# Autodesk Inventor assembly: X-Gantry Joiner Right V3 Assembly
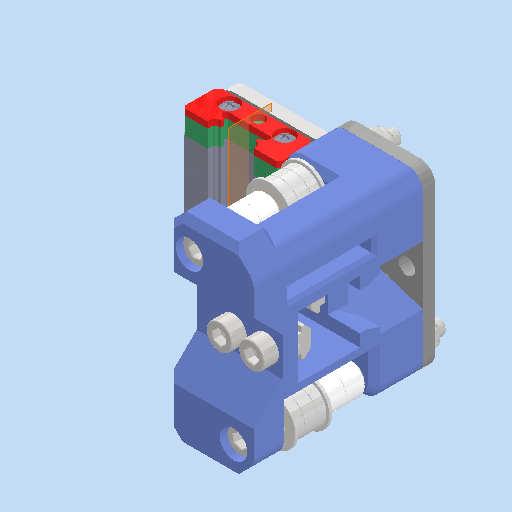
[picture p0: Inventor's stored thumbnail of the model, 512x512]
Saved by Autodesk Inventor 2023.2 (Build 272271000, 271)
## iProperties
Created: 2023-12-06
Part Number: X-Gantry Joiner Right V3 Assembly
Document SubType Name: Assembly
Designer: Nils Bade
Author: Nils Bade
## Documents named in this file (13)
- C:\Users\nilsb\Documents\Inventor\Projektarbeit-Bade\RatRig_Bade\X-Gantry Joiner Right V3 Assembly.iam
- C:\Users\nilsb\Documents\Inventor\Projektarbeit-Bade\RatRig_modified\xy Joiner Right for 4040 V2.ipt
- C:\Users\nilsb\Documents\Inventor\Projektarbeit-Bade\RatRig_modified\MGN15 Linear-Rail-Block.ipt
- C:\Users\nilsb\Documents\Inventor\Projektarbeit-Bade\Schrauben\Cap Head Screw M3x12 v2.ipt
- C:\Users\nilsb\Documents\Inventor\Projektarbeit-Bade\RatRig_Standards\T-Nut - Square type for 2020 - M5 v2.ipt
- C:\Users\nilsb\Documents\Inventor\Projektarbeit-Bade\Schrauben\Cap Head Screw M5x10 v2.ipt
- C:\Users\nilsb\Documents\Inventor\Projektarbeit-Bade\Schrauben\Cap Head Screw M5x60.ipt
- C:\Users\nilsb\Documents\Inventor\Projektarbeit-Bade\RatRig_Standards\Hex Locking Nut - M5 v2.ipt
- C:\Users\nilsb\Documents\Inventor\Projektarbeit-Bade\RatRig_Standards\Mini Precision Shim - 8x5x1mm v2.ipt
- C:\Users\nilsb\Documents\Inventor\Projektarbeit-Bade\RatRig_Standards\Ball Bearing - F695ZZ v1.ipt
- C:\Users\nilsb\Documents\Inventor\Projektarbeit-Bade\RatRig_Standards\Ball Bearing - 695ZZ v1.ipt
- C:\Users\nilsb\Documents\Inventor\Projektarbeit-Bade\RatRig_Standards\Aluminium Spacer - 6mm v2.ipt
- C:\Users\nilsb\Documents\Inventor\Projektarbeit-Bade\RatRig_modified\XY Joiner Plate for 4040 V1.ipt
## Components (33 placed, 12 different names)
1. xy Joiner Right for 4040 V2:1 — Passend:63, Passend:65, Passend:66, Passend:67, Passend:68, Passend:70, Passend:71, Passend:72, Passend:74, Passend:75, Passend:76, Passend:79, Passend:80, Passend:81, Passend:82
2. XY Joiner Plate for 4040 V1:2
3. MGN15 Linear-Rail-Block:1
4. Cap Head Screw M3x12 v2:1
5. Cap Head Screw M3x12 v2:2
6. Cap Head Screw M3x12 v2:3
7. Cap Head Screw M3x12 v2:4
8. T-Nut - Square type for 2020 - M5 v2:1 — Passend:73, Passend:74
9. T-Nut - Square type for 2020 - M5 v2:2 — Passend:78, Passend:80
10. T-Nut - Square type for 2020 - M5 v2:3 — Passend:77, Passend:79
11. Cap Head Screw M5x10 v2:1 — Passend:75, Passend:78, Passend:82
12. Cap Head Screw M5x10 v2:2 — Passend:76, Passend:77, Passend:81
13. Cap Head Screw M5x60:1 — Passend:63, Passend:66
14. Cap Head Screw M5x60:2 — Passend:67, Passend:70
15. Hex Locking Nut - M5 v2:1
16. Hex Locking Nut - M5 v2:2
17. Mini Precision Shim - 8x5x1mm v2:1
18. Mini Precision Shim - 8x5x1mm v2:2
19. Mini Precision Shim - 8x5x1mm v2:3 — Passend:68
20. Mini Precision Shim - 8x5x1mm v2:4
21. Mini Precision Shim - 8x5x1mm v2:5
22. Mini Precision Shim - 8x5x1mm v2:6 — Passend:65
23. Ball Bearing - F695ZZ v1:1
24. Ball Bearing - F695ZZ v1:2
25. Ball Bearing - F695ZZ v1:3
26. Ball Bearing - F695ZZ v1:4
27. Ball Bearing - 695ZZ v1:1
28. Ball Bearing - 695ZZ v1:2
29. Aluminium Spacer - 6mm v2:1
30. Aluminium Spacer - 6mm v2:2
31. Aluminium Spacer - 6mm v2:3
32. Aluminium Spacer - 6mm v2:4
33. Cap Head Screw M5x10 v2:3 — Passend:71, Passend:72, Passend:73
## Relationships (68: Mate 68)
- [Mate]: Cap Head Screw M5x60:1 ↔ Hex Locking Nut - M5 v2:1
- [Mate]: Cap Head Screw M5x60:2 ↔ Hex Locking Nut - M5 v2:2
- [Mate]: Cap Head Screw M5x60:2 ↔ Mini Precision Shim - 8x5x1mm v2:3
- [Mate]: Cap Head Screw M5x60:2 ↔ Ball Bearing - F695ZZ v1:4
- [Mate]: Mini Precision Shim - 8x5x1mm v2:3 ↔ Ball Bearing - F695ZZ v1:4
- [Mate]: Cap Head Screw M5x60:2 ↔ Ball Bearing - 695ZZ v1:1
- [Mate]: Ball Bearing - F695ZZ v1:4 ↔ Ball Bearing - 695ZZ v1:1
- [Mate]: Cap Head Screw M5x60:2 ↔ Ball Bearing - F695ZZ v1:1
- [Mate]: Ball Bearing - F695ZZ v1:1 ↔ Ball Bearing - 695ZZ v1:1
- [Mate]: Cap Head Screw M5x60:2 ↔ Mini Precision Shim - 8x5x1mm v2:2
- [Mate]: Mini Precision Shim - 8x5x1mm v2:2 ↔ Ball Bearing - F695ZZ v1:1
- [Mate]: Cap Head Screw M5x60:2 ↔ Aluminium Spacer - 6mm v2:1
- [Mate]: Mini Precision Shim - 8x5x1mm v2:2 ↔ Aluminium Spacer - 6mm v2:1
- [Mate]: Cap Head Screw M5x60:2 ↔ Aluminium Spacer - 6mm v2:2
- [Mate]: Aluminium Spacer - 6mm v2:1 ↔ Aluminium Spacer - 6mm v2:2
- [Mate]: Cap Head Screw M5x60:2 ↔ Mini Precision Shim - 8x5x1mm v2:1
- [Mate]: Mini Precision Shim - 8x5x1mm v2:1 ↔ Aluminium Spacer - 6mm v2:2
- [Mate]: Cap Head Screw M5x60:1 ↔ Mini Precision Shim - 8x5x1mm v2:4
- [Mate]: Cap Head Screw M5x60:1 ↔ Ball Bearing - F695ZZ v1:2
- [Mate]: Mini Precision Shim - 8x5x1mm v2:4 ↔ Ball Bearing - F695ZZ v1:2
- [Mate]: Cap Head Screw M5x60:1 ↔ Ball Bearing - 695ZZ v1:2
- [Mate]: Ball Bearing - F695ZZ v1:2 ↔ Ball Bearing - 695ZZ v1:2
- [Mate]: Cap Head Screw M5x60:1 ↔ Ball Bearing - F695ZZ v1:3
- [Mate]: Ball Bearing - F695ZZ v1:3 ↔ Ball Bearing - 695ZZ v1:2
- [Mate]: Cap Head Screw M5x60:1 ↔ Mini Precision Shim - 8x5x1mm v2:5
- [Mate]: Mini Precision Shim - 8x5x1mm v2:5 ↔ Ball Bearing - F695ZZ v1:3
- [Mate]: Cap Head Screw M5x60:1 ↔ Aluminium Spacer - 6mm v2:3
- [Mate]: Mini Precision Shim - 8x5x1mm v2:5 ↔ Aluminium Spacer - 6mm v2:3
- [Mate]: Cap Head Screw M5x60:1 ↔ Aluminium Spacer - 6mm v2:4
- [Mate]: Aluminium Spacer - 6mm v2:3 ↔ Aluminium Spacer - 6mm v2:4
- [Mate]: Cap Head Screw M5x60:1 ↔ Mini Precision Shim - 8x5x1mm v2:6
- [Mate]: Mini Precision Shim - 8x5x1mm v2:6 ↔ Aluminium Spacer - 6mm v2:4
- [Mate]: T-Nut - Square type for 2020 - M5 v2:2 ↔ Cap Head Screw M5x10 v2:1
- [Mate]: T-Nut - Square type for 2020 - M5 v2:3 ↔ Cap Head Screw M5x10 v2:2
- [Mate]: xy Joiner Right for 4040 V2:1 ↔ XY Joiner Plate for 4040 V1:2
- [Mate]: xy Joiner Right for 4040 V2:1 ↔ XY Joiner Plate for 4040 V1:2
- [Mate]: xy Joiner Right for 4040 V2:1 ↔ XY Joiner Plate for 4040 V1:2
- [Mate]: XY Joiner Plate for 4040 V1:2 ↔ MGN15 Linear-Rail-Block:1
- [Mate]: XY Joiner Plate for 4040 V1:2 ↔ MGN15 Linear-Rail-Block:1
- [Mate]: XY Joiner Plate for 4040 V1:2 ↔ MGN15 Linear-Rail-Block:1
- [Mate]: XY Joiner Plate for 4040 V1:2 ↔ Cap Head Screw M3x12 v2:2
- [Mate]: XY Joiner Plate for 4040 V1:2 ↔ Cap Head Screw M3x12 v2:1
- [Mate]: XY Joiner Plate for 4040 V1:2 ↔ Cap Head Screw M3x12 v2:4
- [Mate]: XY Joiner Plate for 4040 V1:2 ↔ Cap Head Screw M3x12 v2:3
- [Mate]: XY Joiner Plate for 4040 V1:2 ↔ Cap Head Screw M3x12 v2:3
- [Mate]: XY Joiner Plate for 4040 V1:2 ↔ Cap Head Screw M3x12 v2:4
- [Mate]: XY Joiner Plate for 4040 V1:2 ↔ Cap Head Screw M3x12 v2:1
- [Mate]: XY Joiner Plate for 4040 V1:2 ↔ Cap Head Screw M3x12 v2:2
- Passend:63 [Mate]: xy Joiner Right for 4040 V2:1 ↔ Cap Head Screw M5x60:1
- [Mate]: XY Joiner Plate for 4040 V1:2 ↔ Hex Locking Nut - M5 v2:1
- Passend:65 [Mate]: xy Joiner Right for 4040 V2:1 ↔ Mini Precision Shim - 8x5x1mm v2:6
- Passend:66 [Mate]: xy Joiner Right for 4040 V2:1 ↔ Cap Head Screw M5x60:1
- Passend:67 [Mate]: xy Joiner Right for 4040 V2:1 ↔ Cap Head Screw M5x60:2
- Passend:68 [Mate]: xy Joiner Right for 4040 V2:1 ↔ Mini Precision Shim - 8x5x1mm v2:3
- [Mate]: XY Joiner Plate for 4040 V1:2 ↔ Hex Locking Nut - M5 v2:2
- Passend:70 [Mate]: xy Joiner Right for 4040 V2:1 ↔ Cap Head Screw M5x60:2
- Passend:71 [Mate]: xy Joiner Right for 4040 V2:1 ↔ Cap Head Screw M5x10 v2:3
- Passend:72 [Mate]: xy Joiner Right for 4040 V2:1 ↔ Cap Head Screw M5x10 v2:3
- Passend:73 [Mate]: T-Nut - Square type for 2020 - M5 v2:1 ↔ Cap Head Screw M5x10 v2:3
- Passend:74 [Mate] (1.8 mm): xy Joiner Right for 4040 V2:1 ↔ T-Nut - Square type for 2020 - M5 v2:1
- Passend:75 [Mate]: xy Joiner Right for 4040 V2:1 ↔ Cap Head Screw M5x10 v2:1
- Passend:76 [Mate]: xy Joiner Right for 4040 V2:1 ↔ Cap Head Screw M5x10 v2:2
- Passend:77 [Mate]: T-Nut - Square type for 2020 - M5 v2:3 ↔ Cap Head Screw M5x10 v2:2
- Passend:78 [Mate]: T-Nut - Square type for 2020 - M5 v2:2 ↔ Cap Head Screw M5x10 v2:1
- Passend:79 [Mate] (1.8 mm): xy Joiner Right for 4040 V2:1 ↔ T-Nut - Square type for 2020 - M5 v2:3
- Passend:80 [Mate] (1.8 mm): xy Joiner Right for 4040 V2:1 ↔ T-Nut - Square type for 2020 - M5 v2:2
- Passend:81 [Mate]: xy Joiner Right for 4040 V2:1 ↔ Cap Head Screw M5x10 v2:2
- Passend:82 [Mate]: xy Joiner Right for 4040 V2:1 ↔ Cap Head Screw M5x10 v2:1
## Named parameters: d25_d36 = 0 mm, d5_d37 = 0 mm, d8_d40 = 0 mm, d9_d42 = 0 mm, d10_d43 = 0 mm, d11_d44 = 0 mm
